# Autodesk Inventor assembly: BOTTOM ASSEMBLY BOX
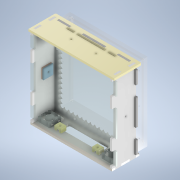
[picture p0: Inventor's stored thumbnail of the model, 180x180]
Saved by Autodesk Inventor 2022.3 (Build 263350030, 350C)
## iProperties
Created: 2021-06-17
Part Number: BOTTOM ASSEMBLY BOX
Document SubType Name: Assembly
Designer: benka
Author: benka
## Documents named in this file (13)
- C:\Users\Ben\OneDrive\Documents\GitHub\OpenMPD_Hardware\Cases\1x1 Rear Pillars\Model\BOTTOM ASSEMBLY BOX.iam
- C:\Users\Ben\OneDrive\Documents\GitHub\OpenMPD_Hardware\Cases\1x1 Rear Pillars\Model\ipt\NewBoardHolder.ipt
- C:\Users\Ben\OneDrive\Documents\GitHub\OpenMPD_Hardware\Cases\1x1 Rear Pillars\Model\ipt\case bottom sides.ipt
- C:\Users\Ben\OneDrive\Documents\GitHub\OpenMPD_Hardware\Cases\1x1 Rear Pillars\Model\ipt\board cover.ipt
- C:\Users\Ben\OneDrive\Documents\GitHub\OpenMPD_Hardware\Cases\1x1 Rear Pillars\Model\ipt\case bottom front.ipt
- C:\Users\Ben\OneDrive\Documents\GitHub\OpenMPD_Hardware\Cases\1x1 Rear Pillars\Model\ipt\case bottom back.ipt
- C:\Users\Ben\OneDrive\Documents\GitHub\OpenMPD_Hardware\Cases\1x1 Rear Pillars\Model\3010fan.iam
- C:\Users\Ben\OneDrive\Documents\GitHub\OpenMPD_Hardware\Cases\1x1 Rear Pillars\Model\ipt\big holder.ipt
- C:\Users\Ben\OneDrive\Documents\GitHub\OpenMPD_Hardware\Cases\1x1 Rear Pillars\Model\ipt\big hex.ipt
- C:\Users\Ben\OneDrive\Documents\GitHub\OpenMPD_Hardware\Cases\1x1 Rear Pillars\Model\ipt\M4 Nut.ipt
- C:\Users\Ben\OneDrive\Documents\GitHub\OpenMPD_Hardware\Cases\1x1 Rear Pillars\Model\ipt\M2 Nut.ipt
- C:\Users\Ben\OneDrive\Documents\GitHub\OpenMPD_Hardware\Cases\1x1 Rear Pillars\Model\ipt\Bottom fabric holder.ipt
- C:\Users\Ben\OneDrive\Documents\GitHub\OpenMPD_Hardware\Cases\1x1 Rear Pillars\Model\ipt\2x 2x M6 Nut Holder.ipt
## Components (27 placed, 12 different names)
1. NewBoardHolder:1 — Mate:81, Mate:82, Mate:83, Mate:84, Mate:85, Mate:86, Mate:87, Mate:88, Mate:89, Mate:92, Mate:94, Flush:4
2. case bottom sides:1 — Flush:3, Mate:87, Mate:88, Mate:89, Insert:12, Angle:2, Mate:100
3. case bottom sides:2 — Mate:84, Mate:85, Mate:86, Insert:11, Angle:1, Mate:101, Flush:13, Mate:107, Mate:109, Mate:110
4. board cover:1 — Mate:107, Mate:108, Mate:109, Mate:110
5. case bottom front:1 — Mate:66, Mate:92, Mate:95, Insert:9, Insert:10, Angle:3, Angle:4
6. case bottom back:1 — Mate:81, Mate:82, Mate:83, Mate:90, Mate:102, Mate:108
7. 3010fan:1 [sub-assembly] — Flush:3, Mate:90, Mate:100
8. 3010fan:2 [sub-assembly] — Mate:101, Mate:102, Flush:13
9. big hex:3 — Mate:96, Flush:5, Flush:6, Angle:3
10. M4 Nut:3 — Insert:5, Insert:10
11. M2 Nut:1
12. M2 Nut:2
13. M2 Nut:3
14. M2 Nut:4
15. Bottom fabric holder:1 — Mate:66, Mate:94, Flush:4, Mate:95
16. 2x 2x M6 Nut Holder:1
17. big holder:5 — Mate:96, Flush:5, Flush:6, Insert:5
18. 2x 2x M6 Nut Holder:3
19. big hex:4 — Angle:1
20. M4 Nut:4 — Insert:11
21. big holder:6
22. big hex:5
23. M4 Nut:5 — Insert:12
24. big holder:7 — Angle:2
25. big hex:6 — Angle:4
26. M4 Nut:6 — Insert:9
27. big holder:8
## Relationships (48: Mate 25, Flush 11, Insert 8, Angle 4)
- Mate:66: case bottom front:1 ↔ Bottom fabric holder:1
- Flush:3 (2 mm): case bottom sides:1 ↔ 3010fan:1
- Mate:81: NewBoardHolder:1 ↔ case bottom back:1
- Mate:82: NewBoardHolder:1 ↔ case bottom back:1
- Mate:83: NewBoardHolder:1 ↔ case bottom back:1
- Mate:84: NewBoardHolder:1 ↔ case bottom sides:2
- Mate:85: NewBoardHolder:1 ↔ case bottom sides:2
- Mate:86: NewBoardHolder:1 ↔ case bottom sides:2
- Mate:87: NewBoardHolder:1 ↔ case bottom sides:1
- Mate:88: NewBoardHolder:1 ↔ case bottom sides:1
- Mate:89: NewBoardHolder:1 ↔ case bottom sides:1
- Mate:90: case bottom back:1 ↔ 3010fan:1
- Mate:92: NewBoardHolder:1 ↔ case bottom front:1
- Mate:94: NewBoardHolder:1 ↔ Bottom fabric holder:1
- Flush:4: NewBoardHolder:1 ↔ Bottom fabric holder:1
- Mate:95: case bottom front:1 ↔ Bottom fabric holder:1
- Mate:96: big hex:3 ↔ big holder:5
- Flush:5: big hex:3 ↔ big holder:5
- Flush:6: big hex:3 ↔ big holder:5
- Insert:5: M4 Nut:3 ↔ big holder:5
- [Mate]: big hex:4 ↔ big holder:6
- [Flush]: big hex:4 ↔ big holder:6
- [Flush]: big hex:4 ↔ big holder:6
- [Insert]: M4 Nut:4 ↔ big holder:6
- [Mate]: big hex:5 ↔ big holder:7
- [Flush]: big hex:5 ↔ big holder:7
- [Flush]: big hex:5 ↔ big holder:7
- [Insert]: M4 Nut:5 ↔ big holder:7
- [Mate]: big hex:6 ↔ big holder:8
- [Flush]: big hex:6 ↔ big holder:8
- [Flush]: big hex:6 ↔ big holder:8
- [Insert]: M4 Nut:6 ↔ big holder:8
- Insert:9: case bottom front:1 ↔ M4 Nut:6
- Insert:10: case bottom front:1 ↔ M4 Nut:3
- Insert:11: case bottom sides:2 ↔ M4 Nut:4
- Insert:12: case bottom sides:1 ↔ M4 Nut:5
- Angle:1 (0 deg): case bottom sides:2 ↔ big hex:4
- Angle:2 (0 deg): case bottom sides:1 ↔ big holder:7
- Angle:3 (0 deg): case bottom front:1 ↔ big hex:3
- Angle:4 (0 deg): case bottom front:1 ↔ big hex:6
- Mate:100 (2 mm): case bottom sides:1 ↔ 3010fan:1
- Mate:101 (2 mm): case bottom sides:2 ↔ 3010fan:2
- Mate:102: case bottom back:1 ↔ 3010fan:2
- Flush:13 (2 mm): case bottom sides:2 ↔ 3010fan:2
- Mate:107: case bottom sides:2 ↔ board cover:1
- Mate:108: board cover:1 ↔ case bottom back:1
- Mate:109: case bottom sides:2 ↔ board cover:1
- Mate:110: case bottom sides:2 ↔ board cover:1
## Named parameters: d153_d148 = 0 mm, d154_d149 = 0 mm, d155_d150 = 0 mm, d156_d152 = 0 mm, d157_d148 = 0 mm, d158_d149 = 0 mm, d159_d150 = 0 mm, d160_d152 = 0 mm, d161_d148 = 0 mm, d162_d149 = 0 mm, d163_d150 = 0 mm, d164_d152 = 0 mm
